# Autodesk Inventor assembly: model 2 comp 2 floor assembly
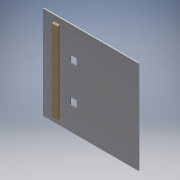
[picture p0: Inventor's stored thumbnail of the model, 180x180]
Saved by Autodesk Inventor 2017 (Build 210142000, 142)
## iProperties
Created: 2017-06-12
Part Number: model 2 comp 2 floor assembly
Document SubType Name: Assembly
Designer: cas7
Author: cas7
## Documents named in this file (4)
- C:\Users\Public\Documents\Autodesk\.desktop-connect\.docstore\guided-tutorial-plugin\INVNTOR\Compartment Modeling\model 2 comp 2 floor assembly.iam
- C:\Users\Public\Documents\Autodesk\.desktop-connect\.docstore\guided-tutorial-plugin\INVNTOR\Compartment Modeling\model 2 comp 2 floor part 1.ipt
- C:\Users\Public\Documents\Autodesk\.desktop-connect\.docstore\guided-tutorial-plugin\INVNTOR\Compartment Modeling\model 2 comp 2 floor part 2.ipt
- C:\Users\Public\Documents\Autodesk\.desktop-connect\.docstore\guided-tutorial-plugin\INVNTOR\Compartment Modeling\holeless 48in 2x4.ipt
## Components (3 placed, 3 different names)
1. model 2 comp 2 floor part 1:1 — Mate:1, Mate:2, Mate:3, Mate:4
2. model 2 comp 2 floor part 2:1 — Mate:1, Mate:2, Mate:5
3. holeless 48in 2x4:1 — Mate:3, Mate:4, Mate:5
## Relationships (5: Mate 5)
- Mate:1: model 2 comp 2 floor part 1:1 ↔ model 2 comp 2 floor part 2:1
- Mate:2: model 2 comp 2 floor part 1:1 ↔ model 2 comp 2 floor part 2:1
- Mate:3 (165.1 mm): model 2 comp 2 floor part 1:1 ↔ holeless 48in 2x4:1
- Mate:4: model 2 comp 2 floor part 1:1 ↔ holeless 48in 2x4:1
- Mate:5 (88.9 mm): model 2 comp 2 floor part 2:1 ↔ holeless 48in 2x4:1
